# Autodesk Inventor assembly: RobotFramewWheelAssembly
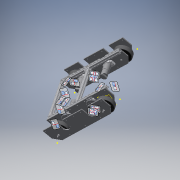
[picture p0: Inventor's stored thumbnail of the model, 180x180]
Saved by Autodesk Inventor 2016 (Build 200138000, 138)
## iProperties
Created: 2016-10-08
Part Number: RobotFramewWheelAssembly
Document SubType Name: Assembly
Designer: RoboticsUser
Author: RoboticsUser
## Documents named in this file (4)
- C:\Robotics\2016-17_CAD\RobotFramewWheelAssembly.iam
- C:\Robotics\2016-17_CAD\WheelAssemblyWFrame.iam
- C:\Robotics\CAD\2015-16\COTSParts\Bosch Extrusion\Bosch 20x20 9 in.ipt
- C:\Robotics\CAD\2015-16\COTSParts\Bosch Extrusion\Gusset 20x20 w screws.ipt
## Components (8 placed, 3 different names)
1. WheelAssemblyWFrame:1 [sub-assembly] — Mate:1, Flush:3, Mate:4, Flush:4
2. WheelAssemblyWFrame:2 [sub-assembly] — Flush:5, Mate:7, Flush:6, Mate:8, Mate:9, Flush:7, Flush:8
3. Bosch 20x20 9 in:1 — Mate:2, Mate:3, Flush:3, Mate:4, Flush:4, Mate:5, Mate:6, Flush:5, Mate:7, Flush:6
4. Gusset 20x20 w screws:1 — Mate:9, Flush:7, Mate:10
5. Gusset 20x20 w screws:2 — Mate:1, Mate:2, Mate:3
6. Gusset 20x20 w screws:3 — Mate:5, Mate:6, Mate:8
7. Gusset 20x20 w screws:4 — Mate:11, Flush:9
8. Bosch 20x20 9 in:2 — Mate:10, Flush:8, Mate:11, Flush:9
## Relationships (18: Mate 11, Flush 7)
- Mate:1: WheelAssemblyWFrame:1 ↔ Gusset 20x20 w screws:2
- Mate:2: Bosch 20x20 9 in:1 ↔ Gusset 20x20 w screws:2
- Mate:3: Bosch 20x20 9 in:1 ↔ Gusset 20x20 w screws:2
- Flush:3: WheelAssemblyWFrame:1 ↔ Bosch 20x20 9 in:1
- Mate:4: WheelAssemblyWFrame:1 ↔ Bosch 20x20 9 in:1
- Flush:4: WheelAssemblyWFrame:1 ↔ Bosch 20x20 9 in:1
- Mate:5: Bosch 20x20 9 in:1 ↔ Gusset 20x20 w screws:3
- Mate:6: Bosch 20x20 9 in:1 ↔ Gusset 20x20 w screws:3
- Flush:5: WheelAssemblyWFrame:2 ↔ Bosch 20x20 9 in:1
- Mate:7: WheelAssemblyWFrame:2 ↔ Bosch 20x20 9 in:1
- Flush:6: WheelAssemblyWFrame:2 ↔ Bosch 20x20 9 in:1
- Mate:8: WheelAssemblyWFrame:2 ↔ Gusset 20x20 w screws:3
- Mate:9: WheelAssemblyWFrame:2 ↔ Gusset 20x20 w screws:1
- Flush:7: WheelAssemblyWFrame:2 ↔ Gusset 20x20 w screws:1
- Mate:10: Gusset 20x20 w screws:1 ↔ Bosch 20x20 9 in:2
- Flush:8: WheelAssemblyWFrame:2 ↔ Bosch 20x20 9 in:2
- Mate:11: Gusset 20x20 w screws:4 ↔ Bosch 20x20 9 in:2
- Flush:9: Gusset 20x20 w screws:4 ↔ Bosch 20x20 9 in:2
